# Autodesk Inventor assembly: Frez No,3
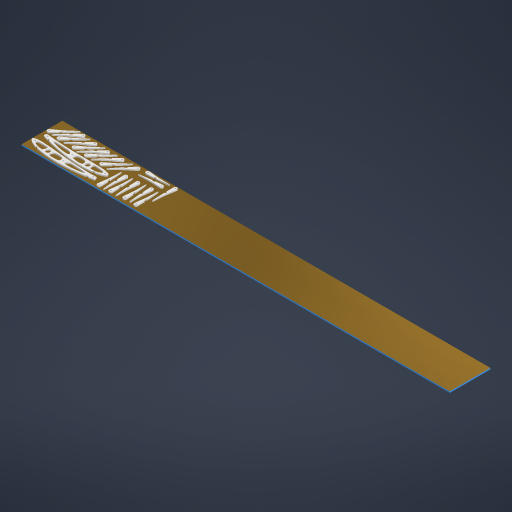
[picture p0: Inventor's stored thumbnail of the model, 512x512]
Saved by Autodesk Inventor 2023 (Build 270158000, 158)
## iProperties
Created: 2023-04-30
Part Number: Frez No,3
Document SubType Name: Assembly
Designer: szykr
Author: szykr
## Documents named in this file (4)
- D:\Folder Instalacyjny\GitHub Pliki\Solaris\new model\Frez_zebra\Frez No,3.iam
- D:\Folder Instalacyjny\GitHub Pliki\Solaris\new model\Frez_zebra\Balsa(95x1000x3).ipt
- D:\Folder Instalacyjny\GitHub Pliki\Solaris\new model\Żebro z lotką.ipt
- D:\Folder Instalacyjny\GitHub Pliki\Solaris\new model\Lotka.ipt
## Components (23 placed, 3 different names)
1. Balsa(95x1000x3):1 — Mate:1, Mate:2, Mate:3, Mate:4, Mate:5, Mate:6, Mate:7, Mate:8, Mate:9, Mate:10, Mate:11, Mate:12, Mate:13, Mate:14, Mate:15, Mate:16, Mate:17, Mate:18, Mate:19, Mate:20, Mate:21, Mate:22
2. Żebro z lotką:1 — Mate:2
3. Żebro z lotką:2 — Mate:1
4. Lotka:1 — Mate:3
5. Lotka:2 — Mate:4
6. Lotka:3 — Mate:5
7. Lotka:4 — Mate:6
8. Lotka:5 — Mate:7
9. Lotka:6 — Mate:8
10. Lotka:7 — Mate:9
11. Lotka:8 — Mate:10
12. Lotka:9 — Mate:11
13. Lotka:10 — Mate:12
14. Lotka:11 — Mate:13
15. Lotka:12 — Mate:14
16. Lotka:13 — Mate:15
17. Lotka:14 — Mate:16
18. Lotka:15 — Mate:17
19. Lotka:16 — Mate:18
20. Lotka:17 — Mate:19
21. Lotka:18 — Mate:20
22. Lotka:19 — Mate:21
23. Lotka:20 — Mate:22
## Relationships (22: Mate 22)
- Mate:1: Balsa(95x1000x3):1 ↔ Żebro z lotką:2
- Mate:2: Balsa(95x1000x3):1 ↔ Żebro z lotką:1
- Mate:3: Balsa(95x1000x3):1 ↔ Lotka:1
- Mate:4: Balsa(95x1000x3):1 ↔ Lotka:2
- Mate:5: Balsa(95x1000x3):1 ↔ Lotka:3
- Mate:6: Balsa(95x1000x3):1 ↔ Lotka:4
- Mate:7: Balsa(95x1000x3):1 ↔ Lotka:5
- Mate:8: Balsa(95x1000x3):1 ↔ Lotka:6
- Mate:9: Balsa(95x1000x3):1 ↔ Lotka:7
- Mate:10: Balsa(95x1000x3):1 ↔ Lotka:8
- Mate:11: Balsa(95x1000x3):1 ↔ Lotka:9
- Mate:12: Balsa(95x1000x3):1 ↔ Lotka:10
- Mate:13: Balsa(95x1000x3):1 ↔ Lotka:11
- Mate:14: Balsa(95x1000x3):1 ↔ Lotka:12
- Mate:15: Balsa(95x1000x3):1 ↔ Lotka:13
- Mate:16: Balsa(95x1000x3):1 ↔ Lotka:14
- Mate:17: Balsa(95x1000x3):1 ↔ Lotka:15
- Mate:18: Balsa(95x1000x3):1 ↔ Lotka:16
- Mate:19: Balsa(95x1000x3):1 ↔ Lotka:17
- Mate:20: Balsa(95x1000x3):1 ↔ Lotka:18
- Mate:21: Balsa(95x1000x3):1 ↔ Lotka:19
- Mate:22: Balsa(95x1000x3):1 ↔ Lotka:20
